# Autodesk Inventor assembly: My Chassy
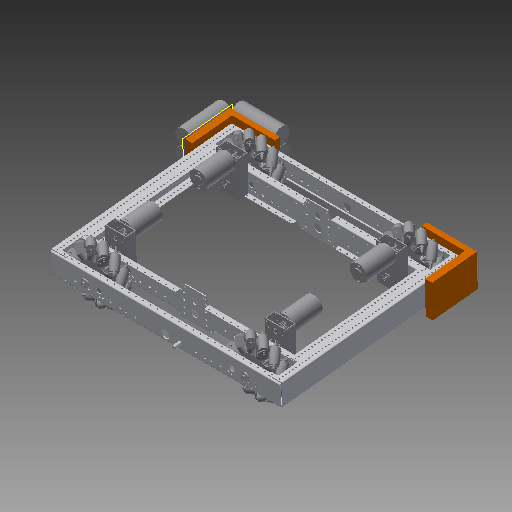
[picture p0: Inventor's stored thumbnail of the model, 512x512]
Saved by Autodesk Inventor 2018 (Build 220112000, 112)
## iProperties
Created: 2016-01-10
Part Number: My Chassy
Document SubType Name: Assembly
Designer: Applefamily
Author: Applefamily
## Documents named in this file (8)
- C:\Users\Apple\Documents\Inventor\2018 PowerUp\2016_Files_2018_Mod\Assembly\My Chassy.iam
- C:\Users\Apple\Documents\Inventor\2018 PowerUp\2016_Files_2018_Mod\Assembly\DriveSide.iam
- C:\Users\Apple\Documents\Inventor\2018 PowerUp\2016_Files_2018_Mod\Assembly\Imported Components\Ground.ipt
- C:\Users\Apple\Documents\Inventor\2018 PowerUp\2016_Files_2018_Mod\Assembly\Imported Components\My2 am-2953 AM14U2 End Sheet Square.ipt.ipt
- C:\Users\Apple\Documents\Inventor\2018 PowerUp\2016_Files_2018_Mod\Sissor Lift\BumperWood.ipt
- C:\Users\Apple\Documents\Inventor\2018 PowerUp\2016_Files_2018_Mod\Sissor Lift\BumperWood2.ipt
- C:\Users\Apple\Documents\Inventor\2018 PowerUp\2016_Files_2018_Mod\Sissor Lift\Noodles.ipt
- My2 am-2953 AM14U2 End Sheet Square.ipt
## Components (11 placed, 6 different names)
1. DriveSide:1 [sub-assembly] — Cylindrical:1, Cylindrical:2, Mate:1, Mate:2, Mate:3, Rotational:1, Rotational:3, Flush:1, Flush:4, Mate:4, Flush:6
2. DriveSide:2 [sub-assembly] — Cylindrical:1, Cylindrical:2, Rotational:2, Rotational:4
3. Ground:1 — Mate:1, Mate:2, Mate:3
4. My2 am-2953 AM14U2 End Sheet Square.ipt:1 — Rotational:1, Rotational:2, Flush:5
5. My2 am-2953 AM14U2 End Sheet Square.ipt:2 — Rotational:3, Rotational:4
6. BumperWood:1 — Flush:1, Flush:2, Flush:3, Flush:4
7. BumperWood2:1 — Flush:2, Flush:3
8. BumperWood:2 — Flush:5, Mate:4, Flush:6, Flush:7, Mate:5, Flush:8
9. BumperWood2:2 — Flush:7, Mate:5, Flush:8, Flush:9, Mate:6
10. Noodles:1 — Flush:10
11. Noodles:2 — Mate:6
## Relationships (22: Flush 10, Mate 6, RevoluteJoint 4, CylindricalJoint 2)
- Cylindrical:1: DriveSide:1 ↔ DriveSide:2
- Cylindrical:2: DriveSide:1 ↔ DriveSide:2
- Mate:1 (101.6 mm): DriveSide:1 ↔ Ground:1
- Mate:2: DriveSide:1 ↔ Ground:1
- Mate:3 (155.1432 mm): DriveSide:1 ↔ Ground:1
- Rotational:1 [RevoluteJoint]: DriveSide:1 ↔ My2 am-2953 AM14U2 End Sheet Square.ipt:1
- Rotational:2 [RevoluteJoint]: DriveSide:2 ↔ My2 am-2953 AM14U2 End Sheet Square.ipt:1
- Rotational:3 [RevoluteJoint]: DriveSide:1 ↔ My2 am-2953 AM14U2 End Sheet Square.ipt:2
- Rotational:4 [RevoluteJoint]: DriveSide:2 ↔ My2 am-2953 AM14U2 End Sheet Square.ipt:2
- Flush:1: DriveSide:1 ↔ BumperWood:1
- Flush:2: BumperWood:1 ↔ BumperWood2:1
- Flush:3: BumperWood:1 ↔ BumperWood2:1
- Flush:4 (-25.4 mm): DriveSide:1 ↔ BumperWood:1
- Flush:5: My2 am-2953 AM14U2 End Sheet Square.ipt:1 ↔ BumperWood:2
- Mate:4: DriveSide:1 ↔ BumperWood:2
- Flush:6 (-25.4 mm): DriveSide:1 ↔ BumperWood:2
- Flush:7: BumperWood:2 ↔ BumperWood2:2
- Mate:5: BumperWood:2 ↔ BumperWood2:2
- Flush:8: BumperWood:2 ↔ BumperWood2:2
- Flush:9: BumperWood2:2
- Flush:10: Noodles:1
- Mate:6 (31.75 mm): BumperWood2:2 ↔ Noodles:2
